# Autodesk Inventor assembly: trebuchet-assembly
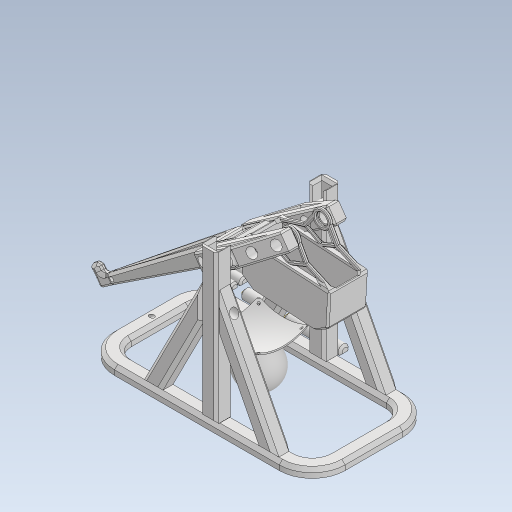
[picture p0: Inventor's stored thumbnail of the model, 512x512]
Saved by Autodesk Inventor 2023 (Build 270158030, 158C)
## iProperties
Created: 2024-12-20
Part Number: trebuchet-assembly
Document SubType Name: Assembly
Designer: Imogen Heard
Author: Imogen Heard
## Documents named in this file (15)
- C:\Users\dheard\Documents\0004-inventor\3D-CAD-main\trebuchet\trebuchet-assembly.iam
- C:\Users\dheard\Documents\0004-inventor\3D-CAD-main\trebuchet\V1_baseplate.ipt
- C:\Users\dheard\Documents\0004-inventor\3D-CAD-main\trebuchet\v1-upright.ipt
- C:\Users\dheard\Documents\0004-inventor\3D-CAD-main\trebuchet\v1-A-frame-a.ipt
- C:\Users\dheard\Documents\0004-inventor\3D-CAD-main\trebuchet\v1-pivot.ipt
- C:\Users\dheard\Documents\0004-inventor\3D-CAD-main\trebuchet\throw-arm.ipt
- C:\Users\dheard\Documents\0004-inventor\3D-CAD-main\trebuchet\v1-counterweight.ipt
- C:\Users\dheard\Documents\0004-inventor\3D-CAD-main\trebuchet\V1-pivot-mirror.ipt
- C:\Users\dheard\Documents\0004-inventor\3D-CAD-main\trebuchet\v1-upright-mirror.ipt
- C:\Users\dheard\Documents\0004-inventor\3D-CAD-main\trebuchet\V1-A-frame-B.ipt
- C:\Users\dheard\Documents\0004-inventor\3D-CAD-main\trebuchet\V1-A-Frame-C.ipt
- C:\Users\dheard\Documents\0004-inventor\3D-CAD-main\trebuchet\V1-A-Frame-D.ipt
- C:\Users\dheard\Documents\0004-inventor\3D-CAD-main\trebuchet\pins.ipt
- C:\Users\dheard\Documents\0004-inventor\3D-CAD-main\trebuchet\bolder.ipt
- C:\Users\dheard\Documents\0004-inventor\3D-CAD-main\trebuchet\sling.ipt
## Components (14 placed, 14 different names)
1. V1_baseplate:1 — Mate:1, Mate:2, Flush:3, Flush:4, Flush:5
2. v1-upright:1
3. v1-A-frame-a:1
4. v1-pivot:1 — Insert:2, Flush:2
5. throw-arm:1 — Insert:1, Flush:1, Insert:2, Flush:2
6. v1-counterweight:1 — Insert:3
7. V1-pivot-mirror:1 — Insert:1, Flush:1, Insert:3, Insert:4
8. v1-upright-mirror:1 — Insert:4, Mate:1, Mate:2, Flush:3
9. V1-A-frame-B:1
10. V1-A-Frame-C:1
11. V1-A-Frame-D:1
12. pins:1 — Flush:4
13. bolder:1 — Flush:5, Flush:6, Flush:7
14. sling:1 — Flush:6, Flush:7
## Relationships (13: Flush 7, Insert 4, Mate 2)
- Insert:1: throw-arm:1 ↔ V1-pivot-mirror:1
- Flush:1: throw-arm:1 ↔ V1-pivot-mirror:1
- Insert:2: v1-pivot:1 ↔ throw-arm:1
- Flush:2: v1-pivot:1 ↔ throw-arm:1
- Insert:3: v1-counterweight:1 ↔ V1-pivot-mirror:1
- Insert:4: V1-pivot-mirror:1 ↔ v1-upright-mirror:1
- Mate:1: V1_baseplate:1 ↔ v1-upright-mirror:1
- Mate:2: V1_baseplate:1 ↔ v1-upright-mirror:1
- Flush:3: V1_baseplate:1 ↔ v1-upright-mirror:1
- Flush:4: V1_baseplate:1 ↔ pins:1
- Flush:5: V1_baseplate:1 ↔ bolder:1
- Flush:6: bolder:1 ↔ sling:1
- Flush:7: bolder:1 ↔ sling:1
